# Autodesk Inventor assembly: MG-Chip Kicker
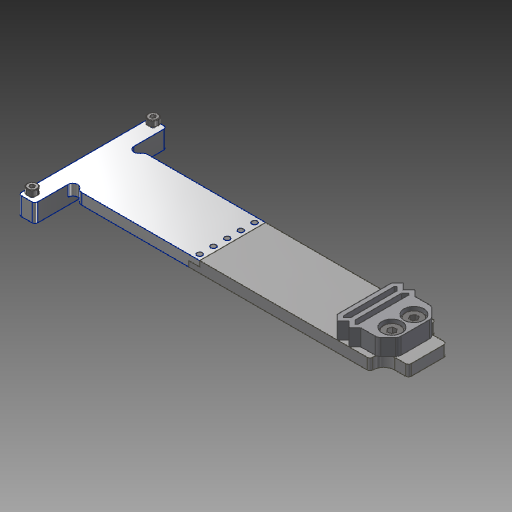
[picture p0: Inventor's stored thumbnail of the model, 512x512]
Saved by Autodesk Inventor 2019.4 (Build 234330000, 330)
## iProperties
Part Number: MG-Chip Kicker
Material: Generisch
Document SubType Name: Assembly
Designer: rYan
Mass: 73.5332 g
Surface Area: 108.095 cm^2
Volume: 14.6899 cm^3
Density: 5.00571 g/cm^3
Author: rYan
## Documents named in this file (7)
- D:\TIGERsGIT\Hardware\mechanik\2020\Inventor\Robot\Kicker\MG-Chip Kicker.iam
- D:\TIGERsGIT\Hardware\mechanik\2020\Inventor\Robot\Kicker\Kicker Chip.ipt
- D:\TIGERsGIT\Hardware\mechanik\2020\Inventor\Robot\Kicker\Kicker Eisen.ipt
- D:\TIGERsGIT\Hardware\mechanik\2020\Inventor\Purchased Parts\DIN EN ISO 2338 - 2 m6 x 4.ipt
- D:\TIGERsGIT\Hardware\mechanik\2020\Inventor\Inhaltscenter\de-DE\ISO 4762(2)\ISO 4762 - M2 x 6ISO.ipt
- D:\TIGERsGIT\Hardware\mechanik\2020\Inventor\Robot\Kicker\Kickerdaempfer.ipt
- D:\TIGERsGIT\Hardware\mechanik\2020\Inventor\Inhaltscenter\de-DE\DIN 7984\DIN 7984 - M4 x 6.ipt
## Components (12 placed, 6 different names)
1. Kicker Chip:1 — Fluchtend:1, Fluchtend:2, Fluchtend:3, Einfügen:1, Passend:1, Einfügen:2, Einfügen:3, Einfügen:4, Einfügen:5, Einfügen:6, Einfügen:9, Einfügen:10
2. Kicker Eisen:1 — Einfügen:1, Passend:1, Einfügen:13, Passend:2
3. DIN EN ISO 2338 - 2 m6 x 4:1 — Einfügen:2
4. DIN EN ISO 2338 - 2 m6 x 4:2 — Einfügen:3
5. DIN EN ISO 2338 - 2 m6 x 4:3 — Einfügen:4
6. DIN EN ISO 2338 - 2 m6 x 4:4 — Einfügen:5
7. DIN EN ISO 2338 - 2 m6 x 4:5 — Einfügen:6
8. ISO 4762 M2 x 6:1 — Einfügen:10
9. ISO 4762 M2 x 6:2 — Einfügen:9
10. Kickerdaempfer:1 — Einfügen:13, Passend:2
11. DIN 7984 M4 x 6:1
12. DIN 7984 M4 x 6:2
## Relationships (16: Insert 11, Flush 3, Mate 2)
- Fluchtend:1 [Flush]: Kicker Chip:1
- Fluchtend:2 [Flush]: Kicker Chip:1
- Fluchtend:3 [Flush]: Kicker Chip:1
- Einfügen:1 [Insert]: Kicker Chip:1 ↔ Kicker Eisen:1
- Passend:1 [Mate]: Kicker Chip:1 ↔ Kicker Eisen:1
- Einfügen:2 [Insert]: Kicker Chip:1 ↔ DIN EN ISO 2338 - 2 m6 x 4:1
- Einfügen:3 [Insert]: Kicker Chip:1 ↔ DIN EN ISO 2338 - 2 m6 x 4:2
- Einfügen:4 [Insert]: Kicker Chip:1 ↔ DIN EN ISO 2338 - 2 m6 x 4:3
- Einfügen:5 [Insert]: Kicker Chip:1 ↔ DIN EN ISO 2338 - 2 m6 x 4:4
- Einfügen:6 [Insert]: Kicker Chip:1 ↔ DIN EN ISO 2338 - 2 m6 x 4:5
- Einfügen:9 [Insert] (1 mm): Kicker Chip:1 ↔ ISO 4762 M2 x 6:2
- Einfügen:10 [Insert] (1 mm): Kicker Chip:1 ↔ ISO 4762 M2 x 6:1
- [Insert]: Kickerdaempfer:1 ↔ DIN 7984 M4 x 6:2
- [Insert]: Kickerdaempfer:1 ↔ DIN 7984 M4 x 6:1
- Einfügen:13 [Insert]: Kicker Eisen:1 ↔ Kickerdaempfer:1
- Passend:2 [Mate]: Kicker Eisen:1 ↔ Kickerdaempfer:1
